# Autodesk Inventor assembly: FrontWheelForkAssembly
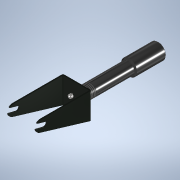
[picture p0: Inventor's stored thumbnail of the model, 180x180]
Saved by Autodesk Inventor 2022.2 (Build 262287000, 287)
## iProperties
Created: 2022-04-13
Part Number: FrontWheelForkAssembly
Document SubType Name: Assembly
Designer: foriw
Author: foriw
## Documents named in this file (5)
- H:\inventor ting\Mekatronik beercart git\Beercart CAD\Workspaces\Workspace\FrontWheelForkAssembly.iam
- H:\inventor ting\Mekatronik beercart git\Beercart CAD\Workspaces\Workspace\Solid2.ipt
- H:\inventor ting\Mekatronik beercart git\Beercart CAD\Workspaces\Workspace\Solid3.ipt
- H:\inventor ting\Mekatronik beercart git\Beercart CAD\Libraries\Content Center Files\en-US\ISO 4762(2)\ISO 4762 - M5 x 12ISO.ipt
- H:\inventor ting\Mekatronik beercart git\Beercart CAD\Libraries\Content Center Files\en-US\ISO 4762(2)\ISO 4762 - M5 x 8ISO.ipt
## Components (4 placed, 4 different names)
1. Solid2:1 — Mate:1, Mate:3
2. Solid3:1 — Mate:2, Mate:4
3. ISO 4762 M5 x 12:1 — Mate:1, Mate:2
4. ISO 4762 M5 x 8:1 — Mate:3, Mate:4
## Relationships (4: Mate 4)
- Mate:1: Solid2:1 ↔ ISO 4762 M5 x 12:1
- Mate:2: Solid3:1 ↔ ISO 4762 M5 x 12:1
- Mate:3: Solid2:1 ↔ ISO 4762 M5 x 8:1
- Mate:4: Solid3:1 ↔ ISO 4762 M5 x 8:1
